# Autodesk Inventor assembly: matrix
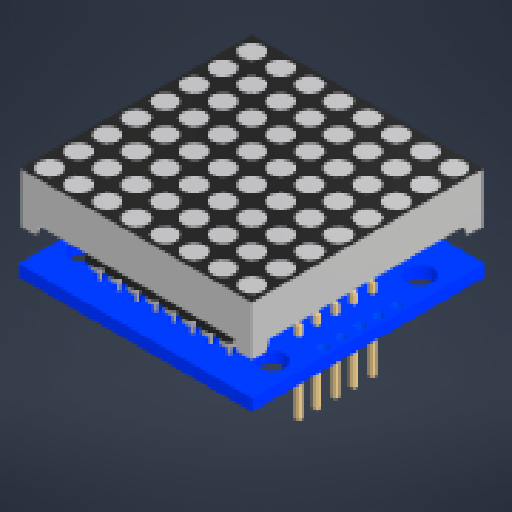
[picture p0: Inventor's stored thumbnail of the model, 512x512]
Saved by Autodesk Inventor 2025.2 (Build 292293000, 293)
## iProperties
Created: 2025-06-28
Part Number: matrix
Document SubType Name: Assembly
Designer: micyg
Author: micyg
## Documents named in this file (6)
- D:\Projects\VirtualPets\VirtualBlob\Mechanical\matrix\matrix.iam
- D:\Projects\VirtualPets\VirtualBlob\Mechanical\matrix\8x_female_rounded_header.ipt
- D:\Projects\VirtualPets\VirtualBlob\Mechanical\matrix\1088AS.ipt
- D:\Projects\VirtualPets\VirtualBlob\Mechanical\matrix\MAX7219.ipt
- D:\Projects\VirtualPets\VirtualBlob\Mechanical\matrix\PCB.ipt
- D:\Projects\VirtualPets\VirtualBlob\Mechanical\matrix\PinHeader_1x05_P2.54mm_Vertical.ipt
## Components (7 placed, 5 different names)
1. 8x_female_rounded_header:1 — Mate:2, Mate:3, Mate:4, Mate:10
2. 1088AS:1 — Mate:10, Mate:11, Mate:12
3. MAX7219:1 — Flush:1, Mate:8, Mate:13
4. PCB:1 — Mate:2, Mate:3, Mate:4, Mate:5, Mate:6, Mate:7, Flush:1, Mate:8, Mate:12, Mate:13, Mate:14, Mate:15, Mate:16, Mate:17, Mate:18, Angle:1, Mate:19, Angle:2
5. 8x_female_rounded_header:2 — Mate:5, Mate:6, Mate:7, Mate:11
6. PinHeader_1x05_P2.54mm_Vertical:1 — Mate:15, Mate:16, Mate:17, Angle:1
7. PinHeader_1x05_P2.54mm_Vertical:2 — Mate:14, Mate:18, Mate:19, Angle:2
## Relationships (20: Mate 17, Angle 2, Flush 1)
- Mate:2: 8x_female_rounded_header:1 ↔ PCB:1
- Mate:3: 8x_female_rounded_header:1 ↔ PCB:1
- Mate:4 (-6.6 mm): 8x_female_rounded_header:1 ↔ PCB:1
- Mate:5: PCB:1 ↔ 8x_female_rounded_header:2
- Mate:6: PCB:1 ↔ 8x_female_rounded_header:2
- Mate:7 (-6.6 mm): PCB:1 ↔ 8x_female_rounded_header:2
- Flush:1 (-8 mm): MAX7219:1 ↔ PCB:1
- Mate:8 (-19 mm): MAX7219:1 ↔ PCB:1
- Mate:10: 8x_female_rounded_header:1 ↔ 1088AS:1
- Mate:11: 1088AS:1 ↔ 8x_female_rounded_header:2
- Mate:12 (-13 mm): 1088AS:1 ↔ PCB:1
- Mate:13: MAX7219:1 ↔ PCB:1
- Mate:14: PCB:1 ↔ PinHeader_1x05_P2.54mm_Vertical:2
- Mate:15: PCB:1 ↔ PinHeader_1x05_P2.54mm_Vertical:1
- Mate:16 (-0.32 mm): PCB:1 ↔ PinHeader_1x05_P2.54mm_Vertical:1
- Mate:17 (-0.32 mm): PCB:1 ↔ PinHeader_1x05_P2.54mm_Vertical:1
- Mate:18 (-0.32 mm): PCB:1 ↔ PinHeader_1x05_P2.54mm_Vertical:2
- Angle:1 (0 deg): PCB:1 ↔ PinHeader_1x05_P2.54mm_Vertical:1
- Mate:19 (-0.32 mm): PCB:1 ↔ PinHeader_1x05_P2.54mm_Vertical:2
- Angle:2 (0 deg): PCB:1 ↔ PinHeader_1x05_P2.54mm_Vertical:2
